# Autodesk Inventor assembly: USB_Soln
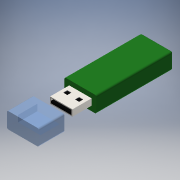
[picture p0: Inventor's stored thumbnail of the model, 180x180]
Saved by Autodesk Inventor 2016 (Build 200138000, 138)
## iProperties
Created: 2017-07-18
Part Number: USB_Soln
Document SubType Name: Assembly
Designer: bobbyl
Author: bobbyl
## Documents named in this file (3)
- C:\Users\bobbyl\Desktop\CAD QuickStart 2017\Lesson 3\USB_Example\USB_Soln.iam
- C:\Users\bobbyl\Desktop\CAD QuickStart 2017\Lesson 3\USB_Example\USB_Stick.ipt
- C:\Users\bobbyl\Desktop\CAD QuickStart 2017\Lesson 3\USB_Example\USB_Cap.ipt
## Components (2 placed, 2 different names)
1. USB_Stick:1 — Mate:1
2. USB_Cap:1 — Mate:1
## Relationships (1: Mate 1)
- Mate:1 (50 mm): USB_Stick:1 ↔ USB_Cap:1
